# Autodesk Inventor assembly: TR1 Actuator
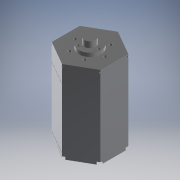
[picture p0: Inventor's stored thumbnail of the model, 180x180]
Saved by Autodesk Inventor 2017 (Build 210142000, 142)
## iProperties
Created: 2018-10-09
Part Number: TR1 Actuator
Document SubType Name: Assembly
Designer: Zach
Author: Zach
## Documents named in this file (13)
- C:\Users\Dell\Documents\GitHub\tr2\Arm Actuator\Arm Actuator.iam
- C:\Users\Dell\Documents\GitHub\tr2\Arm Actuator\TA01.ipt
- C:\Users\Dell\Documents\GitHub\tr2\Arm Actuator\TA02.ipt
- C:\Users\Dell\Documents\GitHub\tr2\Arm Actuator\Arm Actuator\Design Accelerator\Spur Gears2.iam
- C:\Users\Dell\Documents\GitHub\tr2\Arm Actuator\Arm Actuator\Design Accelerator\Spur Gears3.iam
- C:\Users\Dell\Documents\GitHub\tr2\Arm Actuator\TA03.ipt
- C:\Users\Dell\Documents\GitHub\tr2\Arm Actuator\EMS22XXX-D28-LSX.ipt
- C:\Users\Dell\Documents\GitHub\tr2\Arm Actuator\12RPM Gear Motor.ipt
- C:\Users\Dell\Documents\GitHub\tr2\Arm Actuator\Slip Ring.ipt
- C:\Users\Dell\Documents\GitHub\tr2\Arm Actuator\TA06.ipt
- C:\Users\Dell\Documents\GitHub\tr2\Arm Actuator\Bourns ACE 128.ipt
- C:\Users\Dell\Documents\GitHub\tr2\Arm Actuator\Thrust Bearing.ipt
- C:\Users\Dell\Documents\GitHub\tr2\Arm Actuator\6mm Mounting Hub, thin.ipt
## Components (16 placed, 11 different names)
1. TA01:1 — Mate:28, Mate:29, Mate:30
2. TA02:1 — Mate:2, Mate:3, Mate:4, Angle:1, Mate:20, Mate:21, Mate:22, Mate:24, Mate:28, Mate:29, Mate:30, Angle:2, Mate:39, Mate:40, Mate:43, Mate:46, Mate:48, Mate:50, Mate:55, Mate:56, Mate:58, Flush:1
3. TA03:1 — Mate:26, Mate:42, Mate:44, Mate:55
4. TA06:1 — Mate:34, Mate:35, Mate:36
5. Spur Gears:1 [sub-assembly] — Mate:2, Mate:26, Mate:31, Mate:32, Mate:33, Mate:36, Mate:44, Flush:1
6. Spur Gears:2 [sub-assembly] — Mate:3, Mate:4, Mate:51
7. Spur Gears:3 [sub-assembly] — Mate:52, Mate:53, Mate:57, Mate:58
8. Spur Gears:4 [sub-assembly] — Mate:23, Mate:24, Mate:54
9. Thrust Bearing:1 — Mate:42, Mate:43
10. 12RPM Gear Motor:1 — Mate:20, Mate:21, Mate:22, Mate:47
11. EMS22XXX-D28-LSX:1 — Angle:1, Mate:23, Mate:40, Mate:45, Mate:56
12. Bourns ACE 128:1 — Angle:2, Mate:39, Mate:49, Mate:57
13. Slip Ring:1 — Mate:31, Mate:32, Mate:33, Mate:34, Mate:35
14. 6mm Mounting Hub, thin:1 — Mate:45, Mate:46, Mate:54
15. 6mm Mounting Hub, thin:2 — Mate:47, Mate:48, Mate:51
16. 6mm Mounting Hub, thin:3 — Mate:49, Mate:50, Mate:52, Mate:53
## Relationships (40: Mate 37, Angle 2, Flush 1)
- Mate:2: TA02:1 ↔ Spur Gears:1
- Mate:3: TA02:1 ↔ Spur Gears:2
- Mate:4: TA02:1 ↔ Spur Gears:2
- Angle:1 (0 deg): TA02:1 ↔ EMS22XXX-D28-LSX:1
- Mate:20: TA02:1 ↔ 12RPM Gear Motor:1
- Mate:21: TA02:1 ↔ 12RPM Gear Motor:1
- Mate:22: TA02:1 ↔ 12RPM Gear Motor:1
- Mate:23: Spur Gears:4 ↔ EMS22XXX-D28-LSX:1
- Mate:24: TA02:1 ↔ Spur Gears:4
- Mate:26: TA03:1 ↔ Spur Gears:1
- Mate:28: TA01:1 ↔ TA02:1
- Mate:29: TA01:1 ↔ TA02:1
- Mate:30: TA01:1 ↔ TA02:1
- Mate:31: Spur Gears:1 ↔ Slip Ring:1
- Mate:32: Spur Gears:1 ↔ Slip Ring:1
- Mate:33: Spur Gears:1 ↔ Slip Ring:1
- Mate:34: TA06:1 ↔ Slip Ring:1
- Mate:35: TA06:1 ↔ Slip Ring:1
- Mate:36: TA06:1 ↔ Spur Gears:1
- Angle:2 (0 deg): TA02:1 ↔ Bourns ACE 128:1
- Mate:39: TA02:1 ↔ Bourns ACE 128:1
- Mate:40: TA02:1 ↔ EMS22XXX-D28-LSX:1
- Mate:42: TA03:1 ↔ Thrust Bearing:1
- Mate:43: TA02:1 ↔ Thrust Bearing:1
- Mate:44: TA03:1 ↔ Spur Gears:1
- Mate:45: EMS22XXX-D28-LSX:1 ↔ 6mm Mounting Hub, thin:1
- Mate:46: TA02:1 ↔ 6mm Mounting Hub, thin:1
- Mate:47: 12RPM Gear Motor:1 ↔ 6mm Mounting Hub, thin:2
- Mate:48: TA02:1 ↔ 6mm Mounting Hub, thin:2
- Mate:49: Bourns ACE 128:1 ↔ 6mm Mounting Hub, thin:3
- Mate:50: TA02:1 ↔ 6mm Mounting Hub, thin:3
- Mate:51: Spur Gears:2 ↔ 6mm Mounting Hub, thin:2
- Mate:52: Spur Gears:3 ↔ 6mm Mounting Hub, thin:3
- Mate:53: Spur Gears:3 ↔ 6mm Mounting Hub, thin:3
- Mate:54: Spur Gears:4 ↔ 6mm Mounting Hub, thin:1
- Mate:55: TA02:1 ↔ TA03:1
- Mate:56: TA02:1 ↔ EMS22XXX-D28-LSX:1
- Mate:57: Spur Gears:3 ↔ Bourns ACE 128:1
- Mate:58: TA02:1 ↔ Spur Gears:3
- Flush:1: TA02:1 ↔ Spur Gears:1
